# Autodesk Inventor assembly: WedgeBotV3.1
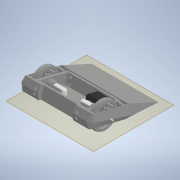
[picture p0: Inventor's stored thumbnail of the model, 180x180]
Saved by Autodesk Inventor 2020 (Build 240168000, 168)
## iProperties
Created: 2023-12-06
Part Number: WedgeBotV3.1
Document SubType Name: Assembly
Designer: smz3rm
Mass: 485.495 g
Surface Area: 1512.57 cm^2
Volume: 447.91 cm^3
Density: 1.08391 g/cm^3
Author: smz3rm
## Documents named in this file (10)
- C:\Users\smz3rm\OneDrive - BP\Documents\DigitalTwin\Models\BattleBot\WedgeBotV3.2.iam
- C:\Users\smz3rm\OneDrive - BP\Documents\DigitalTwin\Models\BattleBot\BodyWedgeWedgeV3.2.ipt
- C:\Users\smz3rm\OneDrive - BP\Documents\DigitalTwin\Models\BattleBot\BodyWedgeBaseV3.2.ipt
- C:\Users\smz3rm\OneDrive - BP\Documents\DigitalTwin\Models\BattleBot\DriveMotorV2.ipt
- C:\Users\smz3rm\OneDrive - BP\Documents\DigitalTwin\Models\BattleBot\BodyWedgeSideV3.2.ipt
- C:\Users\smz3rm\OneDrive - BP\Documents\DigitalTwin\Models\BattleBot\BatteryV1.ipt
- C:\Users\smz3rm\OneDrive - BP\Documents\DigitalTwin\Models\BattleBot\WheelV2.ipt
- C:\Users\smz3rm\OneDrive - BP\Documents\DigitalTwin\Models\BattleBot\FS2A.ipt
- C:\Users\smz3rm\OneDrive - BP\Documents\DigitalTwin\Models\BattleBot\SwitchHolder.ipt
- C:\Users\smz3rm\OneDrive - BP\Documents\DigitalTwin\Models\BattleBot\Switch.ipt
## Components (12 placed, 9 different names)
1. BodyWedgeWedgeV3.2:1 — Mate:1, Mate:2, Mate:3, Mate:4, Mate:5, Mate:6, Mate:11, Mate:22
2. BodyWedgeBaseV3.2:1 — Mate:1, Mate:2, Mate:3, Mate:4, Mate:5, Mate:7, Mate:8, Mate:9, Mate:10, Mate:12, Mate:13, Mate:14, Mate:15, Mate:16, Mate:17, Mate:19, Mate:21, Mate:23, Mate:24, Mate:26, Mate:27, Mate:29, Mate:30, Mate:31, Mate:32, Mate:37, Mate:38, Mate:39, Mate:41, Mate:42
3. DriveMotorV2:1 — Mate:17, Mate:18, Mate:29, Mate:38
4. DriveMotorV2:2 — Mate:16, Mate:20, Mate:30, Mate:39
5. BodyWedgeSideV3.2:1 — Mate:6, Mate:7, Mate:8, Mate:9, Mate:10
6. BodyWedgeSideV3.2:2 — Mate:11, Mate:12, Mate:13, Mate:14, Mate:15
7. BatteryV1:1 — Mate:24, Mate:26, Mate:31
8. WheelV2:1 — Mate:18, Mate:19
9. WheelV2:2 — Mate:20, Mate:21, Tangent:1
10. FS2A:1 — Mate:27, Mate:32, Mate:42
11. SwitchHolder:1 — Mate:34, Mate:35, Mate:37, Mate:40, Mate:41
12. Switch:1 — Mate:34, Mate:35, Mate:40
## Relationships (39: Mate 38, Tangent 1)
- Mate:1: BodyWedgeWedgeV3.2:1 ↔ BodyWedgeBaseV3.2:1
- Mate:2: BodyWedgeWedgeV3.2:1 ↔ BodyWedgeBaseV3.2:1
- Mate:3: BodyWedgeWedgeV3.2:1 ↔ BodyWedgeBaseV3.2:1
- Mate:4: BodyWedgeWedgeV3.2:1 ↔ BodyWedgeBaseV3.2:1
- Mate:5: BodyWedgeWedgeV3.2:1 ↔ BodyWedgeBaseV3.2:1
- Mate:6: BodyWedgeWedgeV3.2:1 ↔ BodyWedgeSideV3.2:1
- Mate:7: BodyWedgeBaseV3.2:1 ↔ BodyWedgeSideV3.2:1
- Mate:8: BodyWedgeBaseV3.2:1 ↔ BodyWedgeSideV3.2:1
- Mate:9: BodyWedgeBaseV3.2:1 ↔ BodyWedgeSideV3.2:1
- Mate:10: BodyWedgeBaseV3.2:1 ↔ BodyWedgeSideV3.2:1
- Mate:11: BodyWedgeWedgeV3.2:1 ↔ BodyWedgeSideV3.2:2
- Mate:12: BodyWedgeBaseV3.2:1 ↔ BodyWedgeSideV3.2:2
- Mate:13: BodyWedgeBaseV3.2:1 ↔ BodyWedgeSideV3.2:2
- Mate:14: BodyWedgeBaseV3.2:1 ↔ BodyWedgeSideV3.2:2
- Mate:15: BodyWedgeBaseV3.2:1 ↔ BodyWedgeSideV3.2:2
- Mate:16: BodyWedgeBaseV3.2:1 ↔ DriveMotorV2:2
- Mate:17: BodyWedgeBaseV3.2:1 ↔ DriveMotorV2:1
- Mate:18: DriveMotorV2:1 ↔ WheelV2:1
- Mate:19: BodyWedgeBaseV3.2:1 ↔ WheelV2:1
- Mate:20: DriveMotorV2:2 ↔ WheelV2:2
- Mate:21: BodyWedgeBaseV3.2:1 ↔ WheelV2:2
- Mate:22: BodyWedgeWedgeV3.2:1
- Mate:23: BodyWedgeBaseV3.2:1
- Mate:24: BodyWedgeBaseV3.2:1 ↔ BatteryV1:1
- Mate:26: BodyWedgeBaseV3.2:1 ↔ BatteryV1:1
- Mate:27: BodyWedgeBaseV3.2:1 ↔ FS2A:1
- Mate:29: BodyWedgeBaseV3.2:1 ↔ DriveMotorV2:1
- Mate:30: BodyWedgeBaseV3.2:1 ↔ DriveMotorV2:2
- Mate:31: BodyWedgeBaseV3.2:1 ↔ BatteryV1:1
- Mate:32: BodyWedgeBaseV3.2:1 ↔ FS2A:1
- Mate:34: SwitchHolder:1 ↔ Switch:1
- Mate:35: SwitchHolder:1 ↔ Switch:1
- Mate:37: BodyWedgeBaseV3.2:1 ↔ SwitchHolder:1
- Mate:38: BodyWedgeBaseV3.2:1 ↔ DriveMotorV2:1
- Mate:39: BodyWedgeBaseV3.2:1 ↔ DriveMotorV2:2
- Tangent:1: WheelV2:2
- Mate:40: SwitchHolder:1 ↔ Switch:1
- Mate:41: BodyWedgeBaseV3.2:1 ↔ SwitchHolder:1
- Mate:42: BodyWedgeBaseV3.2:1 ↔ FS2A:1
